# Autodesk Inventor assembly: ToggleLatch
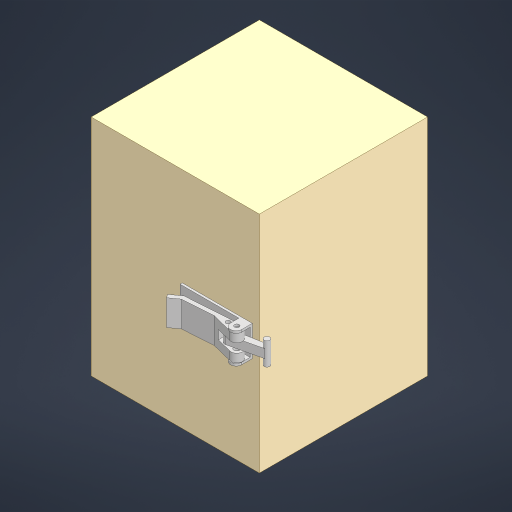
[picture p0: Inventor's stored thumbnail of the model, 512x512]
Saved by Autodesk Inventor 2024.2 (Build 282272000, 272)
## iProperties
Created: 2024-06-05
Part Number: ToggleLatch
Document SubType Name: Assembly
Designer: simon
Author: simon
## Documents named in this file (5)
- C:\Users\simon\Documents\Repositories\GrowBox\hardware\ToggleLatch\ToggleLatch.iam
- C:\Users\simon\Documents\Repositories\GrowBox\hardware\ToggleLatch\Base.ipt
- C:\Users\simon\Documents\Repositories\GrowBox\hardware\ToggleLatch\Lever.ipt
- C:\Users\simon\Documents\Repositories\GrowBox\hardware\ToggleLatch\Latch.ipt
- C:\Users\simon\Documents\Repositories\GrowBox\hardware\ToggleLatch\Corner.ipt
## Components (4 placed, 4 different names)
1. Base:1 — Mate:1, Mate:2, Flush:1, Mate:3, Mate:4, Mate:7, Flush:2, Flush:3
2. Lever:1 — Mate:3, Mate:4, Mate:5, Mate:6
3. Latch:1 — Mate:5, Mate:6
4. Corner:1 — Mate:7, Flush:2, Flush:3
## Relationships (10: Mate 7, Flush 3)
- Mate:1: Base:1
- Mate:2: Base:1
- Flush:1: Base:1
- Mate:3: Base:1 ↔ Lever:1
- Mate:4 (0.1 mm): Base:1 ↔ Lever:1
- Mate:5: Lever:1 ↔ Latch:1
- Mate:6 (0.1 mm): Lever:1 ↔ Latch:1
- Mate:7: Base:1 ↔ Corner:1
- Flush:2 (-5 mm): Base:1 ↔ Corner:1
- Flush:3 (-70 mm): Base:1 ↔ Corner:1
